# Autodesk Inventor assembly: X Axis (1)
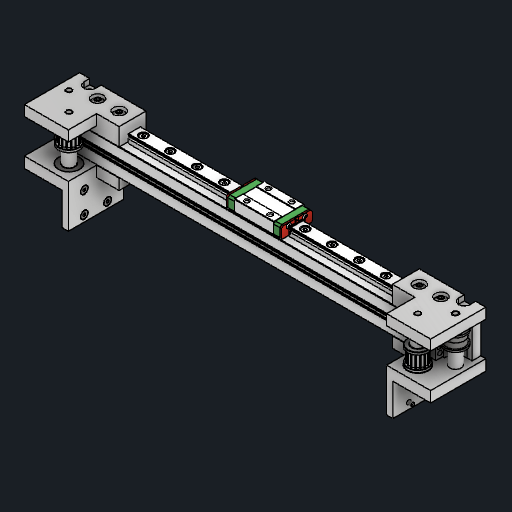
[picture p0: Inventor's stored thumbnail of the model, 512x512]
Saved by Autodesk Inventor 2026.1 (Build 301233020, 233B)
## iProperties
Created: 2025-05-23
Part Number: X Axis (1)
Document SubType Name: Assembly
Designer: Joshua Eah
Author: Joshua Eah
## Documents named in this file (5)
- C:\Users\JoshuaEah\Documents\GitHub\Voron-0\CAD\Tulip - Machined Parts\Tulip Mod Master\X Axis.iam
- C:\Users\JoshuaEah\Documents\GitHub\Voron-0\CAD\Tulip - Machined Parts\Tulip Mod Master\Extrusions.iam
- C:\Users\JoshuaEah\Documents\GitHub\Voron-0\CAD\Tulip - Machined Parts\Tulip Mod Master\MGN7H.iam
- C:\Users\JoshuaEah\Documents\GitHub\Voron-0\CAD\Tulip - Machined Parts\XY Joints\XY Joint Left\XY Joint Left (Tulip).iam
- C:\Users\JoshuaEah\Documents\GitHub\Voron-0\CAD\Tulip - Machined Parts\XY Joints\XY Joint Right\XY Joint Right (Tulip).iam
## Components (4 placed, 4 different names)
1. XY Joint Left (Tulip):1 [sub-assembly]
2. XY Joint Right (Tulip):1 [sub-assembly]
3. Extrusions:1 [sub-assembly]
4. MGN7H:1 [sub-assembly]
## Relationships (2: Mate 2)
- [Mate]: XY Joint Left (Tulip):1 ↔ Extrusions:1
- [Mate]: XY Joint Right (Tulip):1 ↔ Extrusions:1
